# Autodesk Inventor assembly: 強度計算用アセンブリ
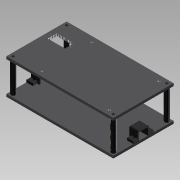
[picture p0: Inventor's stored thumbnail of the model, 180x180]
Saved by Autodesk Inventor 2017 (Build 210142000, 142)
## iProperties
Part Number: 強度計算用アセンブリ
Material: 一般
Document SubType Name: Assembly
Designer: HISAAKI
Mass: 224.314 g
Surface Area: 530.668 cm^2
Volume: 76.964 cm^3
Density: 2.91453 g/cm^3
Author: HISAAKI
## Documents named in this file (25)
- C:\Users\HISAAKI\Documents\LYNCS\CanSat\2017種子島\cansat-structure\強度計算用アセンブリ.iam
- C:\Users\HISAAKI\Documents\LYNCS\CanSat\2017種子島\cansat-structure\基本板.ipt
- C:\Users\HISAAKI\Documents\LYNCS\CanSat\2017種子島\cansat-structure\基本板上.ipt
- C:\Users\HISAAKI\Documents\LYNCS\CanSat\2017種子島\cansat-structure\既成部品\スペーサ.ipt
- C:\Users\HISAAKI\Documents\LYNCS\CanSat\2017種子島\cansat-structure\既成部品\ブラケット.ipt
- C:\Users\HISAAKI\Documents\LYNCS\CanSat\2017種子島\cansat-structure\強度計算用アセンブリ\AIP\FEA\bxpm6i24g.fins
- C:\Users\HISAAKI\Documents\LYNCS\CanSat\2017種子島\cansat-structure\強度計算用アセンブリ\AIP\FEA\bxpm6i3og.fsat
- C:\Users\HISAAKI\Documents\LYNCS\CanSat\2017種子島\cansat-structure\強度計算用アセンブリ\AIP\FEA\bxpm6i3pc.ftes
- C:\Users\HISAAKI\Documents\LYNCS\CanSat\2017種子島\cansat-structure\強度計算用アセンブリ\AIP\FEA\bxpm6i3pc.fwiz
- C:\Users\HISAAKI\Documents\LYNCS\CanSat\2017種子島\cansat-structure\強度計算用アセンブリ\AIP\FEA\bxpm6i5pc.fmsh
- C:\Users\HISAAKI\Documents\LYNCS\CanSat\2017種子島\cansat-structure\強度計算用アセンブリ\AIP\FEA\bxpm6i5pd.fres
- C:\Users\HISAAKI\Documents\LYNCS\CanSat\2017種子島\cansat-structure\強度計算用アセンブリ\AIP\FEA\bxpn6e7r4.fins
- C:\Users\HISAAKI\Documents\LYNCS\CanSat\2017種子島\cansat-structure\強度計算用アセンブリ\AIP\FEA\bxpn6e8kg.fsat
- C:\Users\HISAAKI\Documents\LYNCS\CanSat\2017種子島\cansat-structure\強度計算用アセンブリ\AIP\FEA\bxpn6e8lc.ftes
- C:\Users\HISAAKI\Documents\LYNCS\CanSat\2017種子島\cansat-structure\強度計算用アセンブリ\AIP\FEA\bxpn6e8lc.fwiz
- C:\Users\HISAAKI\Documents\LYNCS\CanSat\2017種子島\cansat-structure\強度計算用アセンブリ\AIP\FEA\bxpn6eef4.fmsh
- C:\Users\HISAAKI\Documents\LYNCS\CanSat\2017種子島\cansat-structure\強度計算用アセンブリ\AIP\FEA\bxpn6eeg0.fres
- C:\Users\HISAAKI\Documents\LYNCS\CanSat\2017種子島\cansat-structure\強度計算用アセンブリ\AIP\FEA\bxpn6efwg.fmsh
- C:\Users\HISAAKI\Documents\LYNCS\CanSat\2017種子島\cansat-structure\強度計算用アセンブリ\AIP\FEA\bxpn6eg9s.fres
- C:\Users\HISAAKI\Documents\LYNCS\CanSat\2017種子島\cansat-structure\強度計算用アセンブリ\AIP\FEA\bzqt9g0io.fins
- C:\Users\HISAAKI\Documents\LYNCS\CanSat\2017種子島\cansat-structure\強度計算用アセンブリ\AIP\FEA\bzqt9g4lc.fsat
- C:\Users\HISAAKI\Documents\LYNCS\CanSat\2017種子島\cansat-structure\強度計算用アセンブリ\AIP\FEA\bzqt9g4lc.ftes
- C:\Users\HISAAKI\Documents\LYNCS\CanSat\2017種子島\cansat-structure\強度計算用アセンブリ\AIP\FEA\bzqt9g4m8.fwiz
- C:\Users\HISAAKI\Documents\LYNCS\CanSat\2017種子島\cansat-structure\強度計算用アセンブリ\AIP\FEA\bzqt9gb28.fmsh
- C:\Users\HISAAKI\Documents\LYNCS\CanSat\2017種子島\cansat-structure\強度計算用アセンブリ\AIP\FEA\bzqt9gb40.fres
## Components (8 placed, 4 different names)
1. 基本板:1 — メイト:1, メイト:2, メイト:3, メイト:4, メイト:5, メイト:6, メイト:7, メイト:8, メイト:14, メイト:15, メイト:16, メイト:17, メイト:18, メイト:19
2. 基本板上:1 — メイト:9, メイト:10, メイト:11, メイト:12, メイト:13
3. スペーサ:1 — メイト:1, メイト:2, メイト:9
4. スペーサ:2 — メイト:3, メイト:6, メイト:10
5. スペーサ:3 — メイト:4, メイト:7, メイト:11
6. スペーサ:4 — メイト:5, メイト:8, メイト:12, メイト:13
7. ブラケット:1 — メイト:14, メイト:15, メイト:16
8. ブラケット:2 — メイト:17, メイト:18, メイト:19
## Relationships (19: Mate 19)
- メイト:1 [Mate]: 基本板:1 ↔ スペーサ:1
- メイト:2 [Mate]: 基本板:1 ↔ スペーサ:1
- メイト:3 [Mate]: 基本板:1 ↔ スペーサ:2
- メイト:4 [Mate]: 基本板:1 ↔ スペーサ:3
- メイト:5 [Mate]: 基本板:1 ↔ スペーサ:4
- メイト:6 [Mate]: 基本板:1 ↔ スペーサ:2
- メイト:7 [Mate]: 基本板:1 ↔ スペーサ:3
- メイト:8 [Mate]: 基本板:1 ↔ スペーサ:4
- メイト:9 [Mate]: 基本板上:1 ↔ スペーサ:1
- メイト:10 [Mate]: 基本板上:1 ↔ スペーサ:2
- メイト:11 [Mate]: 基本板上:1 ↔ スペーサ:3
- メイト:12 [Mate]: 基本板上:1 ↔ スペーサ:4
- メイト:13 [Mate]: 基本板上:1 ↔ スペーサ:4
- メイト:14 [Mate]: 基本板:1 ↔ ブラケット:1
- メイト:15 [Mate]: 基本板:1 ↔ ブラケット:1
- メイト:16 [Mate]: 基本板:1 ↔ ブラケット:1
- メイト:17 [Mate]: 基本板:1 ↔ ブラケット:2
- メイト:18 [Mate]: 基本板:1 ↔ ブラケット:2
- メイト:19 [Mate]: 基本板:1 ↔ ブラケット:2
## Named parameters: sa_3 = -10000, sa_4 = -1.1e-12, sa_5 = 2.7e-12, sa_0 = 5000, sa_1 = 6000, sa_2 = 3000, sa_6 = 75000, sa_7 = 75000
note: some values were not read from the file. Shown as the stored number, unit unknown: "sa_3", "sa_4", "sa_5", "sa_0", "sa_1", "sa_2", "sa_6", "sa_7".
